# Autodesk Inventor assembly: EjeRueda
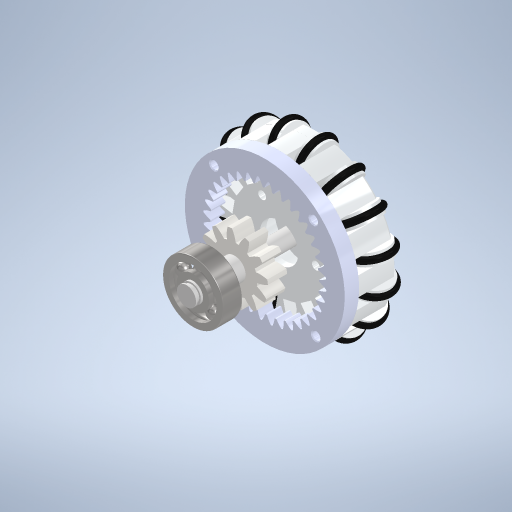
[picture p0: Inventor's stored thumbnail of the model, 512x512]
Saved by Autodesk Inventor 2023 (Build 270158000, 158)
## iProperties
Created: 2022-09-09
Part Number: EjeRueda
Document SubType Name: Assembly
Designer: Lab. de Manufactura
Author: Lab. de Manufactura
## Documents named in this file (5)
- C:\Users\hiago.sodre\Downloads\ssl_CAD-main\Model_2XL430-W250-T\EjeRueda.iam
- C:\Users\hiago.sodre\Downloads\ssl_CAD-main\Model_2XL430-W250-T\EjeSmallSize\eje.ipt
- C:\Users\hiago.sodre\Downloads\ssl_CAD-main\Model_2XL430-W250-T\SmallSize\Design Accelerator\Engranaje recto11.ipt
- C:\Users\hiago.sodre\Downloads\ssl_CAD-main\Model_2XL430-W250-T\BS 290 SKF - SKF 626-2RS1.ipt
- C:\Users\hiago.sodre\Downloads\Projeto FURGBOL\MecânicaOld\Roda antiga modificada\RODA MONTADA.iam
## Components (4 placed, 4 different names)
1. eje:1 — Rígido:2, De rotación:1, De rotación:2
2. Engranaje recto1:1 — Rígido:2
3. BS 290 SKF- con dos juntas RS1 SKF 626-2RS1:1 — De rotación:1
4. RODA MONTADA:1 [sub-assembly] — De rotación:2
## Relationships (3: RevoluteJoint 2, WeldJoint 1)
- Rígido:2 [WeldJoint]: eje:1 ↔ Engranaje recto1:1
- De rotación:1 [RevoluteJoint]: eje:1 ↔ BS 290 SKF- con dos juntas RS1 SKF 626-2RS1:1
- De rotación:2 [RevoluteJoint]: eje:1 ↔ RODA MONTADA:1
